# Autodesk Inventor assembly: Scissor Lift
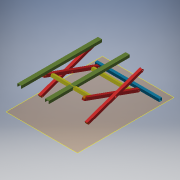
[picture p0: Inventor's stored thumbnail of the model, 180x180]
Saved by Autodesk Inventor 2017 SP1 (Build 210196100, 196)
## iProperties
Created: 2018-01-12
Part Number: Scissor Lift
Document SubType Name: Assembly
Designer: Ben
Author: Ben
## Documents named in this file (6)
- C:\Users\Ben\Desktop\Projects\2018 Robot\Scissor Lift\Scissor Lift.iam
- C:\Users\Ben\Desktop\Projects\2018 Robot\Scissor Lift\Front lift arm.ipt
- C:\Users\Ben\Desktop\Projects\2018 Robot\Scissor Lift\Front lift arm cross.ipt
- C:\Users\Ben\Desktop\Projects\2018 Robot\Scissor Lift\lift wheel.ipt
- C:\Users\Ben\Desktop\Projects\2018 Robot\Scissor Lift\lift rails.ipt
- C:\Users\Ben\Desktop\Projects\2018 Robot\Scissor Lift\lift support arm.ipt
## Components (13 placed, 5 different names)
1. Front lift arm:1 — Insert:6, Mate:3, Flush:13, Mate:4, Insert:8, Flush:14, Mate:8
2. Front lift arm:2 — Insert:5, Mate:1, Flush:10, Flush:11, Mate:2, Insert:7, Flush:12, Mate:4, Mate:5
3. Front lift arm cross:1 — Flush:7, Flush:11, Mate:2
4. Front lift arm cross:2 — Flush:8, Mate:1, Flush:10, Flush:12, Mate:3, Flush:13
5. Front lift arm:3 — Flush:9, Insert:4, Insert:8
6. Front lift arm:4 — Flush:9, Insert:3, Insert:7
7. lift wheel:1 — Insert:3, Tangent:1
8. lift wheel:2 — Insert:4, Tangent:2
9. lift wheel:3 — Insert:6
10. lift wheel:4 — Insert:5
11. lift rails:1
12. lift rails:2
13. lift support arm:1 — Mate:6, Mate:7, Flush:14, Mate:8
## Relationships (24: Flush 8, Mate 8, Insert 6, Tangent 2)
- Flush:7: Front lift arm cross:1
- Flush:8: Front lift arm cross:2
- Flush:9: Front lift arm:3 ↔ Front lift arm:4
- Insert:3 (1.5875 mm): Front lift arm:4 ↔ lift wheel:1
- Insert:4 (1.5875 mm): Front lift arm:3 ↔ lift wheel:2
- Insert:5 (1.5875 mm): Front lift arm:2 ↔ lift wheel:4
- Insert:6 (1.5875 mm): Front lift arm:1 ↔ lift wheel:3
- Mate:1: Front lift arm:2 ↔ Front lift arm cross:2
- Flush:10: Front lift arm:2 ↔ Front lift arm cross:2
- Flush:11: Front lift arm:2 ↔ Front lift arm cross:1
- Mate:2 (50.8 mm): Front lift arm:2 ↔ Front lift arm cross:1
- Insert:7 (4.7625 mm): Front lift arm:2 ↔ Front lift arm:4
- Flush:12 (63.5 mm): Front lift arm:2 ↔ Front lift arm cross:2
- Mate:3: Front lift arm:1 ↔ Front lift arm cross:2
- Flush:13: Front lift arm:1 ↔ Front lift arm cross:2
- Mate:4: Front lift arm:1 ↔ Front lift arm:2
- Insert:8 (4.7625 mm): Front lift arm:1 ↔ Front lift arm:3
- Tangent:1: lift wheel:1
- Tangent:2: lift wheel:2
- Mate:5 (12.7 mm): Front lift arm:2
- Mate:6: lift support arm:1
- Mate:7: lift support arm:1
- Flush:14 (-25.4 mm): Front lift arm:1 ↔ lift support arm:1
- Mate:8 (14.2875 mm): Front lift arm:1 ↔ lift support arm:1
